# Autodesk Inventor assembly: V4 Assembly
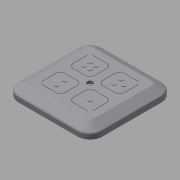
[picture p0: Inventor's stored thumbnail of the model, 180x180]
Saved by Autodesk Inventor 2020 (Build 240168000, 168)
## iProperties
Created: 2020-01-10
Part Number: V4 Assembly
Document SubType Name: Assembly
Designer: user
Author: user
## Documents named in this file (5)
- D:\Documents\Github\Arduino-MiLightHub_switch\3D\V4 Assembly.iam
- D:\Documents\Github\Arduino-MiLightHub_switch\3D\V4 dual in wall.ipt
- D:\Documents\Github\Arduino-MiLightHub_switch\3D\V4 dual.ipt
- D:\Documents\Github\Arduino-MiLightHub_switch\3D\V4 In wall.ipt
- D:\Documents\Github\Arduino-MiLightHub_switch\3D\V4.ipt
## Components (4 placed, 4 different names)
1. V4 dual in wall:1 — Flush:1, Mate:1, Mate:2, Mate:3
2. V4 dual:1 — Flush:1, Mate:1, Mate:2, Flush:2, Flush:3
3. V4:1 — Mate:3, Flush:2, Flush:3, Mate:4, Angle:1, Flush:4
4. V4 In wall:1 — Mate:4, Angle:1, Flush:4
## Relationships (9: Flush 4, Mate 4, Angle 1)
- Flush:1: V4 dual in wall:1 ↔ V4 dual:1
- Mate:1: V4 dual in wall:1 ↔ V4 dual:1
- Mate:2: V4 dual in wall:1 ↔ V4 dual:1
- Mate:3: V4 dual in wall:1 ↔ V4:1
- Flush:2: V4 dual:1 ↔ V4:1
- Flush:3: V4 dual:1 ↔ V4:1
- Mate:4: V4:1 ↔ V4 In wall:1
- Angle:1 (0 deg): V4:1 ↔ V4 In wall:1
- Flush:4: V4:1 ↔ V4 In wall:1
